# Autodesk Inventor assembly: x-aXIS-aSSEMBLY
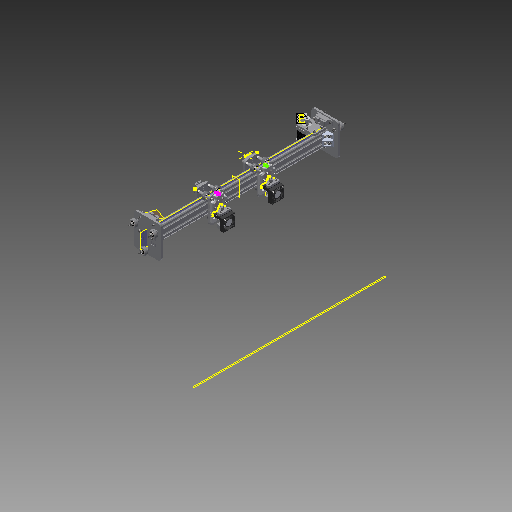
[picture p0: Inventor's stored thumbnail of the model, 512x512]
Saved by Autodesk Inventor 2017 (Build 210142000, 142)
## iProperties
Created: 2016-07-20
Part Number: x-aXIS-aSSEMBLY
Document SubType Name: Assembly
Designer: User
Author: User
## Documents named in this file (34)
- C:\All INVENTOR\SL-Inventor\SL-Beast 3D Printer\x-aXIS-aSSEMBLY.iam
- C:\All INVENTOR\SL-Inventor\SL-Beast 3D Printer\X-Axis-End-Plate.ipt
- C:\All INVENTOR\SL-Inventor\SL-Beast 3D Printer\Makerslide 580mm.ipt
- C:\All INVENTOR\SL-Inventor\SL-Beast 3D Printer\DelrinY-Wheel-Top.iam
- C:\All INVENTOR\SL-Inventor\SL-Beast 3D Printer\DelrinY-Wheel-Bottom.iam
- C:\All INVENTOR\SL-Inventor\SL-Beast 3D Printer\2020corner-assmbly.iam
- C:\All INVENTOR\SL-Inventor\SL-Beast 3D Printer\en-US\ANSI B18.3.1M(6)\ANSI B18.3.1M - M5x0.8 x 10(1).ipt
- C:\All INVENTOR\SL-Inventor\SL-Beast 3D Printer\M5 Tee Nut.ipt
- C:\All INVENTOR\SL-Inventor\SL-Beast 3D Printer\M5 Tee Nut_CPY.ipt
- C:\All INVENTOR\SL-Inventor\SL-Beast 3D Printer\en-US\ANSI B18.3.1M(6)\ANSI B18.3.1M - M5x0.8 x 25(1).ipt
- C:\All INVENTOR\SL-Inventor\SL-Beast 3D Printer\Washer.ipt
- C:\All INVENTOR\SL-Inventor\SL-Beast 3D Printer\Flanged Bearing.ipt
- C:\All INVENTOR\SL-Inventor\SL-Beast 3D Printer\Flanged Bearing_CPY.ipt
- C:\All INVENTOR\SL-Inventor\SL-Beast 3D Printer\en-US\ANSI B 18.2.4.1 M(1)\ANSI B 18.2.4.1 M - M4 x 0.7Style 1.ipt
- C:\All INVENTOR\SL-Inventor\SL-Beast 3D Printer\en-US\ANSI B18.3.1M(6)\ANSI B18.3.1M - M3x0.5 x 16(1).ipt
- C:\All INVENTOR\SL-Inventor\SL-Beast 3D Printer\X-Idler_MIR.ipt
- C:\All INVENTOR\SL-Inventor\SL-Beast 3D Printer\en-US\ANSI B18.16.3M(2)\ANSI B18.16.3M - Property Class 5 and 10 - Metric M3 x 0.5 Metal Type.ipt
- C:\All INVENTOR\SL-Inventor\SL-Beast 3D Printer\X-Axis-End-Plate_MIR.ipt
- C:\All INVENTOR\SL-Inventor\SL-Beast 3D Printer\DelrinY-Wheel-Top_MIR.iam
- C:\All INVENTOR\SL-Inventor\SL-Beast 3D Printer\DelrinY-Wheel-Bottom_MIR.iam
- C:\All INVENTOR\SL-Inventor\SL-Beast 3D Printer\Y Belt Clamp_MIR1.ipt
- C:\All INVENTOR\SL-Inventor\SL-Beast 3D Printer\2020corner-assmbly_MIR2.iam
- C:\All INVENTOR\SL-Inventor\SL-Beast 3D Printer\2020corner-assmbly_MIR2_MIR.iam
- C:\All INVENTOR\SL-Inventor\SL-Beast 3D Printer\Z Motor Mount LC.ipt
- C:\All INVENTOR\SL-Inventor\SL-Beast 3D Printer\M5 Tee Nut-Generic.ipt
- C:\All INVENTOR\SL-Inventor\SL-Beast 3D Printer\M5 Tee Nut-Generic_CPY.ipt
- C:\All INVENTOR\SL-Inventor\SL-Beast 3D Printer\M1173041- NEMA 17.ipt
- C:\All INVENTOR\SL-Inventor\SL-Beast 3D Printer\M3 Washer.ipt
- C:\All INVENTOR\SL-Inventor\SL-Beast 3D Printer\en-US\ANSI B18.3.1M(6)\ANSI B18.3.1M - M3x0.5 x 12(1).ipt
- C:\All INVENTOR\SL-Inventor\SL-Beast 3D Printer\GT2_20tooth.ipt
- C:\All INVENTOR\SL-Inventor\SL-Beast 3D Printer\en-US\ANSI B18.3.6M(05)\ANSI B18.3.6M - M3x0.5 x 5(1).ipt
- C:\All INVENTOR\SL-Inventor\SL-Beast 3D Printer\Hotend Mount Assembly.iam
- C:\All INVENTOR\SL-Inventor\SL-Beast 3D Printer\Hotend Mount Assembly_MIR.iam
- C:\All INVENTOR\SL-Inventor\SL-Beast 3D Printer\Y Belt Clamp.ipt
## Components (53 placed, 33 different names)
1. X-Axis-End-Plate:1 — Mate:1, Mate:2, Mate:3, Mate:4, Mate:5, Mate:6, Mate:7, Flush:2, Flush:3, Insert:4, Insert:5, Mate:47, Flush:19, Mate:71, Flush:21
2. Makerslide 580mm:1 — Mate:1, Mate:8, Mate:9, Flush:1, Flush:2, Mate:15, Mate:17, Flush:7, Flush:8, Flush:9, Mate:45, Flush:10, Flush:12, Mate:56, Flush:16, Mate:59, Mate:67, Mate:68
3. DelrinY-Wheel-Top:1 [sub-assembly] — Mate:3, Mate:5
4. DelrinY-Wheel-Top:2 [sub-assembly] — Mate:2, Mate:4
5. DelrinY-Wheel-Bottom:1 [sub-assembly] — Mate:6, Mate:7
6. Forged Socket Head Cap Screw - Metric M5x0.8 x 10:1 — Mate:14, Mate:29, Mate:30
7. Forged Socket Head Cap Screw - Metric M5x0.8 x 10:2 — Mate:16, Mate:28, Mate:31
8. M5 Tee Nut:1 — Mate:14, Mate:15
9. M5 Tee Nut_CPY:1 — Mate:16, Mate:17
10. Forged Socket Head Cap Screw - Metric M5x0.8 x 25:1 — Mate:19, Mate:21, Mate:35, Mate:36
11. Washer:1 — Mate:18, Mate:32, Mate:33
12. Flanged Bearing:1 — Mate:18, Mate:19, Mate:20, Mate:33, Mate:34, Mate:35
13. Flanged Bearing_CPY:1 — Mate:20, Mate:21, Insert:3
14. Hex Nut Metric M4 x 0.7:1 — Insert:3
15. Forged Socket Head Cap Screw - Metric M3x0.5 x 16:1 — Mate:72
16. Forged Socket Head Cap Screw - Metric M3x0.5 x 16:2
17. X-Idler_MIR:1 — Flush:7, Mate:28, Mate:29, Mate:30, Mate:31, Mate:32, Mate:34, Mate:36
18. Prevailing Torque Type Hex Nut - Steel Metric Property Class 5 and 10 - Metric M3 x 0.5 Metal Type:1 — Insert:4
19. Prevailing Torque Type Hex Nut - Steel Metric Property Class 5 and 10 - Metric M3 x 0.5 Metal Type:2 — Insert:5
20. X-Axis-End-Plate_MIR:1 — Mate:37, Mate:38, Mate:39, Mate:40, Mate:41, Mate:42, Insert:6, Insert:7, Mate:59, Flush:19, Mate:65, Mate:66, Mate:69, Flush:21
21. DelrinY-Wheel-Top_MIR:1 [sub-assembly] — Mate:37, Mate:38
22. DelrinY-Wheel-Top_MIR:2 [sub-assembly] — Mate:39, Mate:40
23. DelrinY-Wheel-Bottom_MIR:1 [sub-assembly] — Mate:41, Mate:42
24. Forged Socket Head Cap Screw - Metric M3x0.5 x 16:3 — Mate:70, Mate:74, Mate:75
25. Forged Socket Head Cap Screw - Metric M3x0.5 x 16:4 — Mate:73, Mate:76
26. Prevailing Torque Type Hex Nut - Steel Metric Property Class 5 and 10 - Metric M3 x 0.5 Metal Type:3 — Insert:6, Mate:74
27. Prevailing Torque Type Hex Nut - Steel Metric Property Class 5 and 10 - Metric M3 x 0.5 Metal Type:4 — Insert:7, Mate:73
28. Y Belt Clamp_MIR1:1
29. 2020corner-assmbly_MIR2:1 [sub-assembly] — Mate:65, Mate:67, Flush:20
30. 2020corner-assmbly_MIR2_MIR:1 [sub-assembly] — Mate:66, Mate:68, Flush:20
31. Z Motor Mount LC:1 — Mate:45, Mate:47, Insert:8, Mate:50, Mate:51, Mate:52, Mate:53, Flush:12, Flush:13
32. Forged Socket Head Cap Screw - Metric M5x0.8 x 10:3 — Insert:8, Mate:48
33. M5 Tee Nut-Generic:1 — Flush:10, Mate:48, Flush:11
34. Forged Socket Head Cap Screw - Metric M5x0.8 x 10:4 — Mate:49, Mate:50, Mate:51
35. M5 Tee Nut-Generic_CPY:1 — Mate:49, Flush:11
36. M1173041- NEMA 17:1 — Mate:52, Mate:53, Flush:15, Mate:57
37. Forged Socket Head Cap Screw - Metric M3x0.5 x 12:1 — Insert:9
38. Forged Socket Head Cap Screw - Metric M3x0.5 x 12:2 — Insert:10
39. Forged Socket Head Cap Screw - Metric M3x0.5 x 12:3 — Insert:11
40. Forged Socket Head Cap Screw - Metric M3x0.5 x 12:4 — Insert:12
41. GT2_20tooth:1 — Mate:57, Mate:58
42. Hotend Mount Assembly:1 [sub-assembly] — Mate:56, Flush:16, Flush:17, Flush:18
43. Hotend Mount Assembly_MIR:1 [sub-assembly] — Flush:17, Flush:18
44. Y Belt Clamp:1 — Mate:69, Mate:70, Mate:75, Mate:76
45. Y Belt Clamp:2 — Mate:71, Mate:72
46. 2020corner-assmbly:1 [sub-assembly] — Mate:8, Mate:9, Flush:1, Flush:3
47. 2020corner-assmbly:2 [sub-assembly]
48. M3 Washer:1 — Flush:13, Insert:9
49. M3 Washer:2 — Insert:12
50. M3 Washer:3 — Insert:10
51. M3 Washer:4 — Insert:11
52. Forged Hexagon Socket Set Screw - Flat Point - Metric M3x0.5 x 5:1 — Flush:15, Mate:58
53. Forged Hexagon Socket Set Screw - Flat Point - Metric M3x0.5 x 5:2
## Component patterns: (2 elements, first: 2020corner-assmbly:1), (4 elements, first: M3 Washer:1), (2 elements, first: Forged Hexagon Socket Set Screw - Flat Point - Metric M3x0.5 x 5:1)
## Relationships (83: Mate 56, Flush 17, Insert 10)
- Mate:1: X-Axis-End-Plate:1 ↔ Makerslide 580mm:1
- Mate:2: X-Axis-End-Plate:1 ↔ DelrinY-Wheel-Top:2
- Mate:3: X-Axis-End-Plate:1 ↔ DelrinY-Wheel-Top:1
- Mate:4: X-Axis-End-Plate:1 ↔ DelrinY-Wheel-Top:2
- Mate:5: X-Axis-End-Plate:1 ↔ DelrinY-Wheel-Top:1
- Mate:6: X-Axis-End-Plate:1 ↔ DelrinY-Wheel-Bottom:1
- Mate:7: X-Axis-End-Plate:1 ↔ DelrinY-Wheel-Bottom:1
- Mate:8: Makerslide 580mm:1 ↔ 2020corner-assmbly:1
- Mate:9 (1.5 mm): Makerslide 580mm:1 ↔ 2020corner-assmbly:1
- Flush:1: Makerslide 580mm:1 ↔ 2020corner-assmbly:1
- Flush:2 (27 mm): X-Axis-End-Plate:1 ↔ Makerslide 580mm:1
- Flush:3 (16 mm): X-Axis-End-Plate:1 ↔ 2020corner-assmbly:1
- Mate:14: Forged Socket Head Cap Screw - Metric M5x0.8 x 10:1 ↔ M5 Tee Nut:1
- Mate:15: Makerslide 580mm:1 ↔ M5 Tee Nut:1
- Mate:16: Forged Socket Head Cap Screw - Metric M5x0.8 x 10:2 ↔ M5 Tee Nut_CPY:1
- Mate:17: Makerslide 580mm:1 ↔ M5 Tee Nut_CPY:1
- Mate:18: Washer:1 ↔ Flanged Bearing:1
- Mate:19: Forged Socket Head Cap Screw - Metric M5x0.8 x 25:1 ↔ Flanged Bearing:1
- Mate:20: Flanged Bearing:1 ↔ Flanged Bearing_CPY:1
- Mate:21: Forged Socket Head Cap Screw - Metric M5x0.8 x 25:1 ↔ Flanged Bearing_CPY:1
- Insert:3: Flanged Bearing_CPY:1 ↔ Hex Nut Metric M4 x 0.7:1
- Flush:7: Makerslide 580mm:1 ↔ X-Idler_MIR:1
- Mate:28: Forged Socket Head Cap Screw - Metric M5x0.8 x 10:2 ↔ X-Idler_MIR:1
- Mate:29: Forged Socket Head Cap Screw - Metric M5x0.8 x 10:1 ↔ X-Idler_MIR:1
- Mate:30: Forged Socket Head Cap Screw - Metric M5x0.8 x 10:1 ↔ X-Idler_MIR:1
- Mate:31: Forged Socket Head Cap Screw - Metric M5x0.8 x 10:2 ↔ X-Idler_MIR:1
- Mate:32: Washer:1 ↔ X-Idler_MIR:1
- Mate:33: Washer:1 ↔ Flanged Bearing:1
- Mate:34: Flanged Bearing:1 ↔ X-Idler_MIR:1
- Mate:35: Forged Socket Head Cap Screw - Metric M5x0.8 x 25:1 ↔ Flanged Bearing:1
- Mate:36: Forged Socket Head Cap Screw - Metric M5x0.8 x 25:1 ↔ X-Idler_MIR:1
- Insert:4: X-Axis-End-Plate:1 ↔ Prevailing Torque Type Hex Nut - Steel Metric Property Class 5 and 10 - Metric M3 x 0.5 Metal Type:1
- Insert:5: X-Axis-End-Plate:1 ↔ Prevailing Torque Type Hex Nut - Steel Metric Property Class 5 and 10 - Metric M3 x 0.5 Metal Type:2
- Flush:8 (-290 mm): Makerslide 580mm:1
- Mate:37: X-Axis-End-Plate_MIR:1 ↔ DelrinY-Wheel-Top_MIR:1
- Mate:38: X-Axis-End-Plate_MIR:1 ↔ DelrinY-Wheel-Top_MIR:1
- Mate:39: X-Axis-End-Plate_MIR:1 ↔ DelrinY-Wheel-Top_MIR:2
- Mate:40: X-Axis-End-Plate_MIR:1 ↔ DelrinY-Wheel-Top_MIR:2
- Mate:41: X-Axis-End-Plate_MIR:1 ↔ DelrinY-Wheel-Bottom_MIR:1
- Mate:42: X-Axis-End-Plate_MIR:1 ↔ DelrinY-Wheel-Bottom_MIR:1
- Insert:6: X-Axis-End-Plate_MIR:1 ↔ Prevailing Torque Type Hex Nut - Steel Metric Property Class 5 and 10 - Metric M3 x 0.5 Metal Type:3
- Insert:7: X-Axis-End-Plate_MIR:1 ↔ Prevailing Torque Type Hex Nut - Steel Metric Property Class 5 and 10 - Metric M3 x 0.5 Metal Type:4
- Flush:9 (-10 mm): Makerslide 580mm:1
- Mate:45: Makerslide 580mm:1 ↔ Z Motor Mount LC:1
- Mate:47: X-Axis-End-Plate:1 ↔ Z Motor Mount LC:1
- Insert:8: Z Motor Mount LC:1 ↔ Forged Socket Head Cap Screw - Metric M5x0.8 x 10:3
- Flush:10 (2.5 mm): Makerslide 580mm:1 ↔ M5 Tee Nut-Generic:1
- Mate:48: Forged Socket Head Cap Screw - Metric M5x0.8 x 10:3 ↔ M5 Tee Nut-Generic:1
- Mate:49: Forged Socket Head Cap Screw - Metric M5x0.8 x 10:4 ↔ M5 Tee Nut-Generic_CPY:1
- Mate:50: Z Motor Mount LC:1 ↔ Forged Socket Head Cap Screw - Metric M5x0.8 x 10:4
- Mate:51: Z Motor Mount LC:1 ↔ Forged Socket Head Cap Screw - Metric M5x0.8 x 10:4
- Flush:11: M5 Tee Nut-Generic:1 ↔ M5 Tee Nut-Generic_CPY:1
- Mate:52: Z Motor Mount LC:1 ↔ M1173041- NEMA 17:1
- Mate:53: Z Motor Mount LC:1 ↔ M1173041- NEMA 17:1
- Flush:12 (3.5 mm): Makerslide 580mm:1 ↔ Z Motor Mount LC:1
- Flush:13: Z Motor Mount LC:1 ↔ M3 Washer:1
- Insert:9: Forged Socket Head Cap Screw - Metric M3x0.5 x 12:1 ↔ M3 Washer:1
- Insert:10: Forged Socket Head Cap Screw - Metric M3x0.5 x 12:2 ↔ M3 Washer:3
- Insert:11: Forged Socket Head Cap Screw - Metric M3x0.5 x 12:3 ↔ M3 Washer:4
- Insert:12: Forged Socket Head Cap Screw - Metric M3x0.5 x 12:4 ↔ M3 Washer:2
- Flush:15 (-5 mm): M1173041- NEMA 17:1 ↔ Forged Hexagon Socket Set Screw - Flat Point - Metric M3x0.5 x 5:1
- Mate:56 (5.5 mm): Makerslide 580mm:1 ↔ Hotend Mount Assembly:1
- Flush:16 (-23 mm): Makerslide 580mm:1 ↔ Hotend Mount Assembly:1
- Flush:17: Hotend Mount Assembly:1 ↔ Hotend Mount Assembly_MIR:1
- Flush:18: Hotend Mount Assembly:1 ↔ Hotend Mount Assembly_MIR:1
- Mate:57: M1173041- NEMA 17:1 ↔ GT2_20tooth:1
- Mate:58: GT2_20tooth:1 ↔ Forged Hexagon Socket Set Screw - Flat Point - Metric M3x0.5 x 5:1
- Mate:59: Makerslide 580mm:1 ↔ X-Axis-End-Plate_MIR:1
- Flush:19: X-Axis-End-Plate:1 ↔ X-Axis-End-Plate_MIR:1
- Mate:65: X-Axis-End-Plate_MIR:1 ↔ 2020corner-assmbly_MIR2:1
- Mate:66: X-Axis-End-Plate_MIR:1 ↔ 2020corner-assmbly_MIR2_MIR:1
- Mate:67: Makerslide 580mm:1 ↔ 2020corner-assmbly_MIR2:1
- Mate:68: Makerslide 580mm:1 ↔ 2020corner-assmbly_MIR2_MIR:1
- Flush:20: 2020corner-assmbly_MIR2:1 ↔ 2020corner-assmbly_MIR2_MIR:1
- Mate:69: X-Axis-End-Plate_MIR:1 ↔ Y Belt Clamp:1
- Mate:70: Forged Socket Head Cap Screw - Metric M3x0.5 x 16:3 ↔ Y Belt Clamp:1
- Mate:71: X-Axis-End-Plate:1 ↔ Y Belt Clamp:2
- Mate:72: Forged Socket Head Cap Screw - Metric M3x0.5 x 16:1 ↔ Y Belt Clamp:2
- Flush:21: X-Axis-End-Plate:1 ↔ X-Axis-End-Plate_MIR:1
- Mate:73: Forged Socket Head Cap Screw - Metric M3x0.5 x 16:4 ↔ Prevailing Torque Type Hex Nut - Steel Metric Property Class 5 and 10 - Metric M3 x 0.5 Metal Type:4
- Mate:74: Forged Socket Head Cap Screw - Metric M3x0.5 x 16:3 ↔ Prevailing Torque Type Hex Nut - Steel Metric Property Class 5 and 10 - Metric M3 x 0.5 Metal Type:3
- Mate:75: Forged Socket Head Cap Screw - Metric M3x0.5 x 16:3 ↔ Y Belt Clamp:1
- Mate:76: Forged Socket Head Cap Screw - Metric M3x0.5 x 16:4 ↔ Y Belt Clamp:1
